# Autodesk Inventor assembly: Plate 1
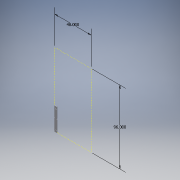
[picture p0: Inventor's stored thumbnail of the model, 180x180]
Saved by Autodesk Inventor 2016 (Build 200138000, 138)
## iProperties
Created: 2016-04-26
Part Number: Plate 1
Document SubType Name: Assembly
Designer: rubenjm
Author: rubenjm
## Documents named in this file (2)
- C:\Users\rubenjm\Documents\To Transfer\2k16 Spring\RME\GGC\V3\Plate 1.iam
- C:\Users\rubenjm\Documents\To Transfer\2k16 Spring\RME\GGC\V3\Arm Base.ipt
## Components (1 placed, 1 different names)
1. Arm Base:1 — Mate:1, Mate:2, Mate:3
## Relationships (3: Mate 3)
- Mate:1: Arm Base:1
- Mate:2: Arm Base:1
- Mate:3: Arm Base:1
